# Autodesk Inventor assembly: NewDUBR
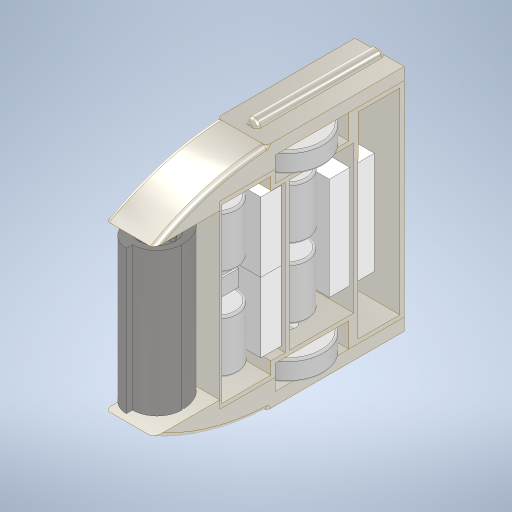
[picture p0: Inventor's stored thumbnail of the model, 512x512]
Saved by Autodesk Inventor 2024.2 (Build 282272000, 272)
## iProperties
Created: 2025-03-01
Part Number: NewDUBR
Document SubType Name: Assembly
Designer: Timofey
Author: Timofey
## Documents named in this file (15)
- C:\Users\Timofey\Documents\NewDUBR.iam
- C:\Users\Timofey\Documents\Деталь1.ipt
- C:\Users\Timofey\Documents\КреплениеБарабана.ipt
- C:\Users\Timofey\Documents\ОсноваКорпуса.ipt
- C:\Users\Timofey\Documents\Колесо.ipt
- C:\Users\Timofey\Documents\МоторКолес.ipt
- C:\Users\Timofey\Documents\Контроллер.ipt
- C:\Users\Timofey\Documents\КонтроллерСпинер.ipt
- C:\Users\Timofey\Documents\Аккумулятор.ipt
- C:\Users\Timofey\Documents\Боковина.ipt
- C:\Users\Timofey\Documents\Inventor\Content Center Files\R2024\ru-RU\GOST 7796-70\Болт M10-6gx60 ГОСТ 7796-70.ipt
- C:\Users\Timofey\Documents\NewDUBR\AIP\FEA\f03xu5juo.fins
- C:\Users\Timofey\Documents\NewDUBR\AIP\FEA\f03xu5jvk.fsat
- C:\Users\Timofey\Documents\NewDUBR\AIP\FEA\f03xu5jvk.ftes
- C:\Users\Timofey\Documents\NewDUBR\AIP\FEA\f03xu5jvk.fwiz
## Components (28 placed, 10 different names)
1. Барабан — Совмещение:6
2. КреплениеБарабана:1 — Совмещение:26, Совмещение:27, Совмещение:28, Совмещение:29, Совмещение:30, Совмещение:31, Совмещение:32, Совмещение:33
3. КреплениеБарабана:2 — Совмещение:6, Совмещение:34, Совмещение:35, Совмещение:36, Совмещение:37, Совмещение:38, Совмещение:39, Совмещение:40, Совмещение:41
4. ОсноваКорпуса:1 — Совмещение:12, Совмещение:13, Совмещение:14, Совмещение:15, Совмещение:16, Совмещение:18, Совмещение:19, Совмещение:20, Совмещение:21, Совмещение:22, Совмещение:23, Совмещение:42, Заподлицо:9, Заподлицо:10, Заподлицо:11, Совмещение:43, Заподлицо:12
5. Колесо:1 — Совмещение:9, С поворотом:1
6. Колесо:2 — Совмещение:10, Цилиндрический:1
7. МоторКолес:1 — Совмещение:10
8. МоторКолес:2 — Совмещение:9
9. МоторКолес:3
10. МоторКолес:4
11. Контроллер:1 — Заподлицо:5, Совмещение:11, Заподлицо:6, Совмещение:13
12. Контроллер:2 — Заподлицо:5, Совмещение:11, Заподлицо:6, Совмещение:12
13. КонтроллерСпинер:1 — Совмещение:14, Совмещение:16, Заподлицо:7, Заподлицо:8, Совмещение:17
14. КонтроллерСпинер:2 — Совмещение:15, Заподлицо:7, Заподлицо:8, Совмещение:17
15. Аккумулятор:1 — Совмещение:18
16. Аккумулятор:2 — Совмещение:19
17. Аккумулятор:3 — Совмещение:20, Совмещение:23
18. Аккумулятор:4 — Совмещение:21, Совмещение:22
19. Боковина:1 — Заподлицо:11, Совмещение:43, Заподлицо:12, С поворотом:1
20. Боковина:2 — Совмещение:42, Заподлицо:9, Заподлицо:10, Цилиндрический:1
21. Болт ГОСТ 7796-70 M10-6gx60:1 — Совмещение:26, Совмещение:27
22. Болт ГОСТ 7796-70 M10-6gx60:2 — Совмещение:28, Совмещение:29
23. Болт ГОСТ 7796-70 M10-6gx60:3 — Совмещение:30, Совмещение:31
24. Болт ГОСТ 7796-70 M10-6gx60:4 — Совмещение:32, Совмещение:33
25. Болт ГОСТ 7796-70 M10-6gx60:5 — Совмещение:34, Совмещение:35
26. Болт ГОСТ 7796-70 M10-6gx60:6 — Совмещение:36, Совмещение:37
27. Болт ГОСТ 7796-70 M10-6gx60:7 — Совмещение:38, Совмещение:39
28. Болт ГОСТ 7796-70 M10-6gx60:8 — Совмещение:40, Совмещение:41
## Relationships (44: Mate 34, Flush 8, CylindricalJoint 1, RevoluteJoint 1)
- Совмещение:6 [Mate]: Барабан ↔ КреплениеБарабана:2
- Совмещение:9 [Mate]: Колесо:1 ↔ МоторКолес:2
- Совмещение:10 [Mate]: Колесо:2 ↔ МоторКолес:1
- Заподлицо:5 [Flush]: Контроллер:1 ↔ Контроллер:2
- Совмещение:11 [Mate] (10 mm): Контроллер:1 ↔ Контроллер:2
- Заподлицо:6 [Flush]: Контроллер:1 ↔ Контроллер:2
- Совмещение:12 [Mate]: ОсноваКорпуса:1 ↔ Контроллер:2
- Совмещение:13 [Mate]: ОсноваКорпуса:1 ↔ Контроллер:1
- Совмещение:14 [Mate]: ОсноваКорпуса:1 ↔ КонтроллерСпинер:1
- Совмещение:15 [Mate]: ОсноваКорпуса:1 ↔ КонтроллерСпинер:2
- Совмещение:16 [Mate]: ОсноваКорпуса:1 ↔ КонтроллерСпинер:1
- Заподлицо:7 [Flush]: КонтроллерСпинер:1 ↔ КонтроллерСпинер:2
- Заподлицо:8 [Flush]: КонтроллерСпинер:1 ↔ КонтроллерСпинер:2
- Совмещение:17 [Mate]: КонтроллерСпинер:1 ↔ КонтроллерСпинер:2
- Совмещение:18 [Mate]: ОсноваКорпуса:1 ↔ Аккумулятор:1
- Совмещение:19 [Mate]: ОсноваКорпуса:1 ↔ Аккумулятор:2
- Совмещение:20 [Mate]: ОсноваКорпуса:1 ↔ Аккумулятор:3
- Совмещение:21 [Mate]: ОсноваКорпуса:1 ↔ Аккумулятор:4
- Совмещение:22 [Mate]: ОсноваКорпуса:1 ↔ Аккумулятор:4
- Совмещение:23 [Mate]: ОсноваКорпуса:1 ↔ Аккумулятор:3
- Совмещение:26 [Mate]: КреплениеБарабана:1 ↔ Болт ГОСТ 7796-70 M10-6gx60:1
- Совмещение:27 [Mate]: КреплениеБарабана:1 ↔ Болт ГОСТ 7796-70 M10-6gx60:1
- Совмещение:28 [Mate]: КреплениеБарабана:1 ↔ Болт ГОСТ 7796-70 M10-6gx60:2
- Совмещение:29 [Mate]: КреплениеБарабана:1 ↔ Болт ГОСТ 7796-70 M10-6gx60:2
- Совмещение:30 [Mate]: КреплениеБарабана:1 ↔ Болт ГОСТ 7796-70 M10-6gx60:3
- Совмещение:31 [Mate]: КреплениеБарабана:1 ↔ Болт ГОСТ 7796-70 M10-6gx60:3
- Совмещение:32 [Mate]: КреплениеБарабана:1 ↔ Болт ГОСТ 7796-70 M10-6gx60:4
- Совмещение:33 [Mate]: КреплениеБарабана:1 ↔ Болт ГОСТ 7796-70 M10-6gx60:4
- Совмещение:34 [Mate]: КреплениеБарабана:2 ↔ Болт ГОСТ 7796-70 M10-6gx60:5
- Совмещение:35 [Mate]: КреплениеБарабана:2 ↔ Болт ГОСТ 7796-70 M10-6gx60:5
- Совмещение:36 [Mate]: КреплениеБарабана:2 ↔ Болт ГОСТ 7796-70 M10-6gx60:6
- Совмещение:37 [Mate]: КреплениеБарабана:2 ↔ Болт ГОСТ 7796-70 M10-6gx60:6
- Совмещение:38 [Mate]: КреплениеБарабана:2 ↔ Болт ГОСТ 7796-70 M10-6gx60:7
- Совмещение:39 [Mate]: КреплениеБарабана:2 ↔ Болт ГОСТ 7796-70 M10-6gx60:7
- Совмещение:40 [Mate]: КреплениеБарабана:2 ↔ Болт ГОСТ 7796-70 M10-6gx60:8
- Совмещение:41 [Mate]: КреплениеБарабана:2 ↔ Болт ГОСТ 7796-70 M10-6gx60:8
- Совмещение:42 [Mate]: ОсноваКорпуса:1 ↔ Боковина:2
- Заподлицо:9 [Flush]: ОсноваКорпуса:1 ↔ Боковина:2
- Заподлицо:10 [Flush]: ОсноваКорпуса:1 ↔ Боковина:2
- Заподлицо:11 [Flush]: ОсноваКорпуса:1 ↔ Боковина:1
- Совмещение:43 [Mate]: ОсноваКорпуса:1 ↔ Боковина:1
- Заподлицо:12 [Flush]: ОсноваКорпуса:1 ↔ Боковина:1
- Цилиндрический:1 [CylindricalJoint]: Колесо:2 ↔ Боковина:2
- С поворотом:1 [RevoluteJoint]: Колесо:1 ↔ Боковина:1
## Named parameters: sa_0 = 500000
note: some values were not read from the file. Shown as the stored number, unit unknown: "sa_0".
